# Autodesk Inventor assembly: LIM
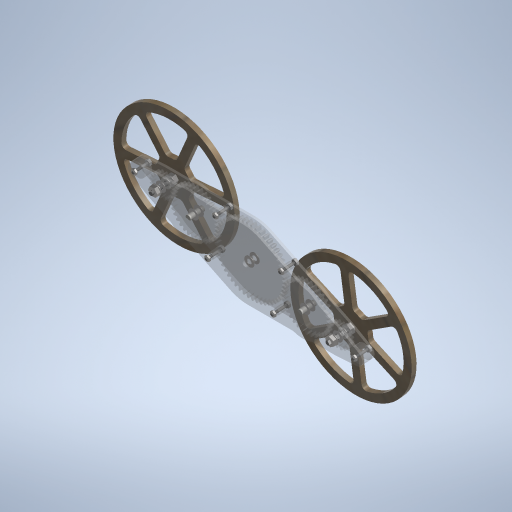
[picture p0: Inventor's stored thumbnail of the model, 512x512]
Saved by Autodesk Inventor 2023 (Build 270158000, 158)
## iProperties
Part Number: LIM
Document SubType Name: Assembly
Designer: Ronan
Author: Ronan
## Documents named in this file (11)
- D:\Libraries\Documents\2023-FYP\Inventor\LIM.iam
- D:\Libraries\Documents\2023-FYP\Inventor\frame.ipt
- D:\Libraries\Documents\2023-FYP\Inventor\Shaft2.ipt
- D:\Libraries\Documents\2023-FYP\Inventor\Assembly\Design Accelerator\Spur Gears3.iam
- D:\Libraries\Documents\2023-FYP\Inventor\standoff1.ipt
- D:\Libraries\Documents\2023-FYP\Inventor\wheel shaft.iam
- D:\Libraries\Documents\2023-FYP\Inventor\Assembly\Design Accelerator\Spur Gear14.ipt
- D:\Libraries\Documents\2023-FYP\Inventor\M5-washer.ipt
- D:\Libraries\Documents\2023-FYP\Inventor\standoff2.ipt
- D:\Libraries\Documents\2023-FYP\Inventor\m3 bolt long.ipt
- D:\Libraries\Documents\2023-FYP\Inventor\M3-nut.ipt
## Components (32 placed, 10 different names)
1. frame:1 — Rotational:1, Cylindrical:1, Mate:11, Mate:12, Mate:15, Mate:17, Mate:18, Cylindrical:4, Mate:33, Mate:34, Mate:51
2. Shaft:2 — Rotational:1, Mate:5, Cylindrical:12, Mate:35
3. Shaft:4 — Cylindrical:1, Rotation:1, Mate:22, Cylindrical:7, Mate:35
4. Spur Gears:1 [sub-assembly] — Mate:5, Rotation:2, Rotation:3, Mate:27, Mate:28, Mate:29, Mate:30, Cylindrical:13
5. standoff1:1 — Mate:11, Mate:14, Mate:16, Mate:17, Mate:18
6. standoff1:2 — Mate:12, Mate:13, Mate:15
7. frame:2 — Mate:13, Mate:14, Mate:16, Cylindrical:2, Cylindrical:3, Cylindrical:8, Cylindrical:9, Cylindrical:10, Cylindrical:11, Mate:25, Mate:26, Mate:36, Mate:37, Mate:38, Mate:40, Mate:41, Mate:42, Mate:43, Mate:44, Mate:45, Mate:46, Mate:47, Mate:48, Mate:49, Mate:50, Mate:58
8. wheel shaft:1 [sub-assembly] — Cylindrical:2, Rotation:3, Mate:26
9. wheel shaft:2 [sub-assembly] — Cylindrical:3, Rotation:1, Mate:25
10. Spur Gear1:1 — Cylindrical:4, Mate:22, Rotation:2, Mate:31, Mate:32
11. M5-washer:3 — Cylindrical:7, Mate:31
12. M5-washer:4 — Cylindrical:8, Mate:32, Mate:33
13. M5-washer:5 — Cylindrical:9, Mate:29
14. M5-washer:6 — Cylindrical:10, Mate:30, Mate:34, Cylindrical:13
15. M5-washer:7 — Cylindrical:11, Mate:27
16. M5-washer:8 — Cylindrical:12, Mate:28
17. standoff2:1 — Mate:36, Mate:40
18. standoff2:2 — Mate:37, Mate:41
19. standoff2:3 — Mate:38, Mate:42
20. standoff2:4 — Mate:43, Mate:44
21. m3 bolt long:1 — Flush:1, Mate:45, Mate:51, Mate:57
22. m3 bolt long:2 — Flush:2, Mate:46, Mate:56
23. m3 bolt long:3 — Flush:3, Flush:5, Mate:48, Mate:54
24. m3 bolt long:4 — Flush:4, Mate:49, Mate:53
25. m3 bolt long:5 — Flush:5, Mate:50, Mate:52
26. m3 bolt long:6 — Flush:1, Flush:2, Flush:3, Flush:4, Mate:47, Mate:55
27. M3-nut:1 — Flush:10, Mate:52
28. M3-nut:2 — Flush:9, Flush:10, Mate:53
29. M3-nut:3 — Flush:8, Flush:9, Mate:54
30. M3-nut:4 — Flush:7, Flush:8, Mate:55
31. M3-nut:5 — Flush:6, Flush:7, Mate:56
32. M3-nut:6 — Flush:6, Mate:57, Mate:58
## Relationships (68: Mate 43, CylindricalJoint 11, Flush 10, RelateRotation 3, RevoluteJoint 1)
- Rotational:1 [RevoluteJoint] (-4.5 mm): frame:1 ↔ Shaft:2
- Cylindrical:1: frame:1 ↔ Shaft:4
- Mate:5: Shaft:2 ↔ Spur Gears:1
- Mate:11: frame:1 ↔ standoff1:1
- Mate:12: frame:1 ↔ standoff1:2
- Mate:13: standoff1:2 ↔ frame:2
- Mate:14: standoff1:1 ↔ frame:2
- Mate:15: frame:1 ↔ standoff1:2
- Mate:16: standoff1:1 ↔ frame:2
- Cylindrical:2: frame:2 ↔ wheel shaft:1
- Mate:17: frame:1 ↔ standoff1:1
- Mate:18: frame:1 ↔ standoff1:1
- Cylindrical:3: frame:2 ↔ wheel shaft:2
- Rotation:1 [RelateRotation] (-0.4848 ul): Shaft:4 ↔ wheel shaft:2
- Cylindrical:4: frame:1 ↔ Spur Gear1:1
- Mate:22: Shaft:4 ↔ Spur Gear1:1
- Rotation:2 [RelateRotation] (-1.5152 ul): Spur Gears:1 ↔ Spur Gear1:1
- Rotation:3 [RelateRotation] (-0.4848 ul): Spur Gears:1 ↔ wheel shaft:1
- Cylindrical:7: Shaft:4 ↔ M5-washer:3
- Cylindrical:8: frame:2 ↔ M5-washer:4
- Cylindrical:9: frame:2 ↔ M5-washer:5
- Cylindrical:10: frame:2 ↔ M5-washer:6
- Cylindrical:11: frame:2 ↔ M5-washer:7
- Cylindrical:12: Shaft:2 ↔ M5-washer:8
- Mate:25: frame:2 ↔ wheel shaft:2
- Mate:26: frame:2 ↔ wheel shaft:1
- Mate:27: Spur Gears:1 ↔ M5-washer:7
- Mate:28: Spur Gears:1 ↔ M5-washer:8
- Mate:29: Spur Gears:1 ↔ M5-washer:5
- Mate:30: Spur Gears:1 ↔ M5-washer:6
- Mate:31: Spur Gear1:1 ↔ M5-washer:3
- Mate:32: Spur Gear1:1 ↔ M5-washer:4
- Mate:33: frame:1 ↔ M5-washer:4
- Mate:34: frame:1 ↔ M5-washer:6
- Cylindrical:13: Spur Gears:1 ↔ M5-washer:6
- Mate:35: Shaft:2 ↔ Shaft:4
- Mate:36: frame:2 ↔ standoff2:1
- Mate:37: frame:2 ↔ standoff2:2
- Mate:38: frame:2 ↔ standoff2:3
- Mate:40: frame:2 ↔ standoff2:1
- Mate:41: frame:2 ↔ standoff2:2
- Mate:42: frame:2 ↔ standoff2:3
- Mate:43: frame:2 ↔ standoff2:4
- Mate:44: frame:2 ↔ standoff2:4
- Flush:1: m3 bolt long:1 ↔ m3 bolt long:6
- Flush:2: m3 bolt long:2 ↔ m3 bolt long:6
- Flush:3: m3 bolt long:3 ↔ m3 bolt long:6
- Flush:4: m3 bolt long:4 ↔ m3 bolt long:6
- Flush:5: m3 bolt long:3 ↔ m3 bolt long:5
- Mate:45: frame:2 ↔ m3 bolt long:1
- Mate:46: frame:2 ↔ m3 bolt long:2
- Mate:47: frame:2 ↔ m3 bolt long:6
- Mate:48: frame:2 ↔ m3 bolt long:3
- Mate:49: frame:2 ↔ m3 bolt long:4
- Mate:50: frame:2 ↔ m3 bolt long:5
- Mate:51: frame:1 ↔ m3 bolt long:1
- Flush:6: M3-nut:5 ↔ M3-nut:6
- Flush:7: M3-nut:4 ↔ M3-nut:5
- Flush:8: M3-nut:3 ↔ M3-nut:4
- Flush:9: M3-nut:2 ↔ M3-nut:3
- Flush:10: M3-nut:1 ↔ M3-nut:2
- Mate:52: m3 bolt long:5 ↔ M3-nut:1
- Mate:53: m3 bolt long:4 ↔ M3-nut:2
- Mate:54: m3 bolt long:3 ↔ M3-nut:3
- Mate:55: m3 bolt long:6 ↔ M3-nut:4
- Mate:56: m3 bolt long:2 ↔ M3-nut:5
- Mate:57: m3 bolt long:1 ↔ M3-nut:6
- Mate:58: frame:2 ↔ M3-nut:6
